# Autodesk Inventor assembly: outside-c-channel_MIR1
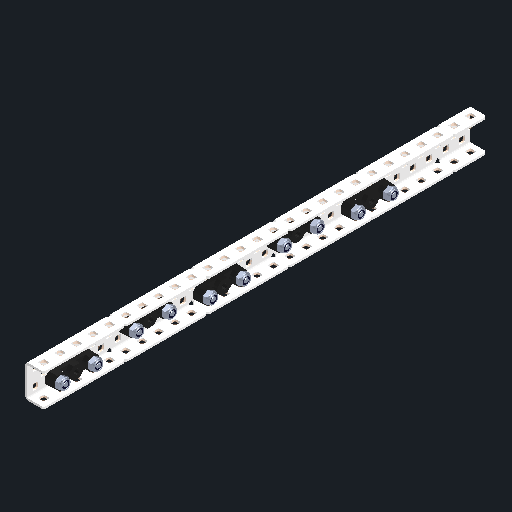
[picture p0: Inventor's stored thumbnail of the model, 512x512]
Saved by Autodesk Inventor 2023 (Build 270158000, 158)
## iProperties
Created: 2023-08-05
Part Number: outside-c-channel_MIR1
Document SubType Name: Assembly
Designer: srbel
Author: srbel
## Documents named in this file (6)
- C:\CAD\OverUnderCAD\Drive\outside-c-channel_MIR1.iam
- C:\CAD\OverUnderCAD\VEX-CAD-Inventor-1.4.0\Structure\C Channel\Aluminum 1x2x1\Alu C 1x2x1x27_MIR1.ipt
- C:\CAD\OverUnderCAD\VEX-CAD-Inventor-1.4.0\Motion\Shaft LS\Bearing Flat_MIR2.ipt
- C:\CAD\OverUnderCAD\VEX-CAD-Inventor-1.4.0\Structure\Hardware\Screw Steel - Star\SScrew Star Threaded .500.ipt
- C:\CAD\OverUnderCAD\VEX-CAD-Inventor-1.4.0\Structure\Hardware\Screw Steel - Star.ipt
- C:\CAD\OverUnderCAD\VEX-CAD-Inventor-1.4.0\Structure\Hardware\Nut Thin Nylock_MIR2.ipt
## Components (26 placed, 4 different names)
1. Alu C 1x2x1x27_MIR1:1 — Insert:2, Insert:1, Insert:4, Insert:3, Insert:6, Insert:5, Insert:8, Insert:7, Insert:22, Insert:21, Insert:23, Insert:24, Insert:25, Insert:26, Insert:27, Insert:28, Insert:29, Insert:30, Insert:31, Insert:32
2. Bearing Flat_MIR2:1 — Insert:2, Insert:1, Insert:41, Insert:42
3. Bearing Flat_MIR2:2 — Insert:4, Insert:3, Insert:39, Insert:40
4. Bearing Flat_MIR2:3 — Insert:6, Insert:5, Insert:37, Insert:38
5. Bearing Flat_MIR2:4 — Insert:8, Insert:7, Insert:35, Insert:36
6. Bearing Flat_MIR2:5 — Insert:22, Insert:21, Insert:33, Insert:34
7. SScrew Star Threaded .500:1 — Insert:23
8. SScrew Star Threaded .500:2 — Insert:24
9. SScrew Star Threaded .500:3 — Insert:25
10. SScrew Star Threaded .500:4 — Insert:26
11. SScrew Star Threaded .500:5 — Insert:27
12. SScrew Star Threaded .500:6 — Insert:28
13. SScrew Star Threaded .500:7 — Insert:29
14. SScrew Star Threaded .500:8 — Insert:30
15. SScrew Star Threaded .500:9 — Insert:31
16. SScrew Star Threaded .500:10 — Insert:32
17. Nut Thin Nylock_MIR2:1 — Insert:33
18. Nut Thin Nylock_MIR2:2 — Insert:34
19. Nut Thin Nylock_MIR2:3 — Insert:35
20. Nut Thin Nylock_MIR2:4 — Insert:36
21. Nut Thin Nylock_MIR2:5 — Insert:37
22. Nut Thin Nylock_MIR2:6 — Insert:38
23. Nut Thin Nylock_MIR2:7 — Insert:39
24. Nut Thin Nylock_MIR2:8 — Insert:40
25. Nut Thin Nylock_MIR2:9 — Insert:41
26. Nut Thin Nylock_MIR2:10 — Insert:42
## Relationships (30: Insert 30)
- Insert:2: Alu C 1x2x1x27_MIR1:1 ↔ Bearing Flat_MIR2:1
- Insert:1: Alu C 1x2x1x27_MIR1:1 ↔ Bearing Flat_MIR2:1
- Insert:4: Alu C 1x2x1x27_MIR1:1 ↔ Bearing Flat_MIR2:2
- Insert:3: Alu C 1x2x1x27_MIR1:1 ↔ Bearing Flat_MIR2:2
- Insert:6: Alu C 1x2x1x27_MIR1:1 ↔ Bearing Flat_MIR2:3
- Insert:5: Alu C 1x2x1x27_MIR1:1 ↔ Bearing Flat_MIR2:3
- Insert:8: Alu C 1x2x1x27_MIR1:1 ↔ Bearing Flat_MIR2:4
- Insert:7: Alu C 1x2x1x27_MIR1:1 ↔ Bearing Flat_MIR2:4
- Insert:22: Alu C 1x2x1x27_MIR1:1 ↔ Bearing Flat_MIR2:5
- Insert:21: Alu C 1x2x1x27_MIR1:1 ↔ Bearing Flat_MIR2:5
- Insert:23: Alu C 1x2x1x27_MIR1:1 ↔ SScrew Star Threaded .500:1
- Insert:24: Alu C 1x2x1x27_MIR1:1 ↔ SScrew Star Threaded .500:2
- Insert:25: Alu C 1x2x1x27_MIR1:1 ↔ SScrew Star Threaded .500:3
- Insert:26: Alu C 1x2x1x27_MIR1:1 ↔ SScrew Star Threaded .500:4
- Insert:27: Alu C 1x2x1x27_MIR1:1 ↔ SScrew Star Threaded .500:5
- Insert:28: Alu C 1x2x1x27_MIR1:1 ↔ SScrew Star Threaded .500:6
- Insert:29: Alu C 1x2x1x27_MIR1:1 ↔ SScrew Star Threaded .500:7
- Insert:30: Alu C 1x2x1x27_MIR1:1 ↔ SScrew Star Threaded .500:8
- Insert:31: Alu C 1x2x1x27_MIR1:1 ↔ SScrew Star Threaded .500:9
- Insert:32: Alu C 1x2x1x27_MIR1:1 ↔ SScrew Star Threaded .500:10
- Insert:33: Bearing Flat_MIR2:5 ↔ Nut Thin Nylock_MIR2:1
- Insert:34: Bearing Flat_MIR2:5 ↔ Nut Thin Nylock_MIR2:2
- Insert:35: Bearing Flat_MIR2:4 ↔ Nut Thin Nylock_MIR2:3
- Insert:36: Bearing Flat_MIR2:4 ↔ Nut Thin Nylock_MIR2:4
- Insert:37: Bearing Flat_MIR2:3 ↔ Nut Thin Nylock_MIR2:5
- Insert:38: Bearing Flat_MIR2:3 ↔ Nut Thin Nylock_MIR2:6
- Insert:39: Bearing Flat_MIR2:2 ↔ Nut Thin Nylock_MIR2:7
- Insert:40: Bearing Flat_MIR2:2 ↔ Nut Thin Nylock_MIR2:8
- Insert:41: Bearing Flat_MIR2:1 ↔ Nut Thin Nylock_MIR2:9
- Insert:42: Bearing Flat_MIR2:1 ↔ Nut Thin Nylock_MIR2:10
